# Autodesk Inventor assembly: Wedge Assembly
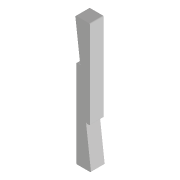
[picture p0: Inventor's stored thumbnail of the model, 180x180]
Saved by Autodesk Inventor 2020 (Build 240168000, 168)
## iProperties
Created: 2020-08-11
Part Number: Wedge Assembly
Document SubType Name: Assembly
Designer: Dan Wikman
Author: Dan Wikman
## Documents named in this file (2)
- C:\Users\Dan Wikman\OneDrive\University Life\2020, Semester 1\METR4900 Honours Thesis\PROTOTYPE V2\Wedge Assembly.iam
- C:\Users\Dan Wikman\OneDrive\University Life\2020, Semester 1\METR4900 Honours Thesis\PROTOTYPE V2\Wedge - V2.ipt
## Components (2 placed, 1 different names)
1. Wedge - V2:1 — Mate:1, Mate:2, Flush:1
2. Wedge - V2:2 — Mate:1, Mate:2, Flush:1
## Relationships (3: Mate 2, Flush 1)
- Mate:1: Wedge - V2:1 ↔ Wedge - V2:2
- Mate:2 (-7 mm): Wedge - V2:1 ↔ Wedge - V2:2
- Flush:1: Wedge - V2:1 ↔ Wedge - V2:2
